# Autodesk Inventor assembly: assembly
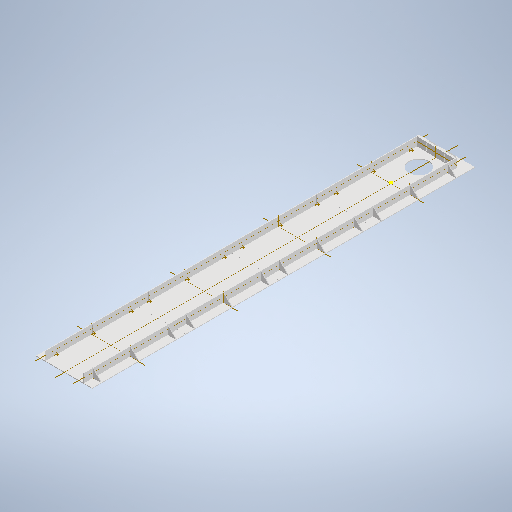
[picture p0: Inventor's stored thumbnail of the model, 512x512]
Saved by Autodesk Inventor 2025 (Build 290162000, 162)
## iProperties
Created: 2024-04-06
Part Number: assembly
Document SubType Name: Assembly
Designer: gmsee
Author: gmsee
## Documents named in this file (6)
- C:\Users\gmsee\OneDrive\바탕 화면\새 폴더\assembly.iam
- C:\Users\gmsee\OneDrive\바탕 화면\새 폴더\end_wall.ipt
- C:\Users\gmsee\OneDrive\바탕 화면\새 폴더\plate_hole.ipt
- C:\Users\gmsee\OneDrive\바탕 화면\새 폴더\plate_middle.ipt
- C:\Users\gmsee\OneDrive\바탕 화면\새 폴더\side_wall.ipt
- C:\Users\gmsee\OneDrive\바탕 화면\새 폴더\supporter.ipt
## Components (39 placed, 5 different names)
1. end_wall:1
2. plate_hole:1 — 플러쉬:1
3. plate_middle:1 — 플러쉬:1, 플러쉬:2
4. side_wall:1
5. supporter:1
6. plate_middle:2 — 플러쉬:2, 플러쉬:3
7. plate_middle:3 — 플러쉬:3
8. supporter:2
9. supporter:3
10. supporter:4
11. supporter:5
12. supporter:6
13. supporter:7
14. supporter:8
15. supporter:9
16. supporter:10
17. supporter:11
18. supporter:12
19. supporter:13
20. supporter:14
21. supporter:15
22. supporter:16
23. supporter:17
24. supporter:18
25. supporter:19
26. supporter:20
27. supporter:21
28. supporter:22
29. supporter:23
30. supporter:24
31. supporter:25
32. supporter:26
33. side_wall:2
34. side_wall:3
35. side_wall:4
36. side_wall:5
37. side_wall:6
38. side_wall:7
39. side_wall:8
## Relationships (3: Flush 3)
- 플러쉬:1 [Flush]: plate_hole:1 ↔ plate_middle:1
- 플러쉬:2 [Flush]: plate_middle:1 ↔ plate_middle:2
- 플러쉬:3 [Flush]: plate_middle:2 ↔ plate_middle:3
